# Autodesk Inventor assembly: Inner_Components
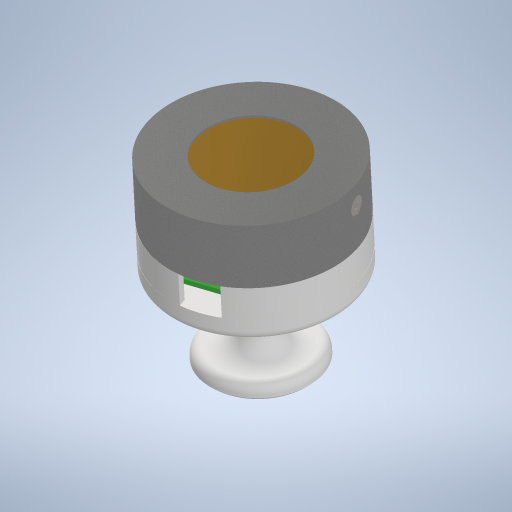
[picture p0: Inventor's stored thumbnail of the model, 512x512]
Saved by Autodesk Inventor 2023 (Build 270158000, 158)
## iProperties
Created: 2023-02-27
Part Number: Inner_Components
Document SubType Name: Assembly
Designer: maste
Author: maste
## Documents named in this file (9)
- C:\Users\maste\Documents\GitHub\Remote-Stethoscope\3D_models\ThonkLabs 1ne\SurfaceContact\Inner_Components.iam
- C:\Users\maste\Documents\GitHub\Remote-Stethoscope\3D_models\ThonkLabs 1ne\SurfaceContact\PiezoMount.ipt
- C:\Users\maste\Documents\GitHub\Remote-Stethoscope\3D_models\ThonkLabs 1ne\SurfaceContact\Piezo.ipt
- C:\Users\maste\Documents\GitHub\Remote-Stethoscope\3D_models\ThonkLabs 1ne\SurfaceContact\Diaphragm_lock.ipt
- C:\Users\maste\Documents\GitHub\Remote-Stethoscope\3D_models\ThonkLabs 1ne\SurfaceContact\holding_socket.ipt
- C:\Users\maste\Documents\GitHub\Remote-Stethoscope\3D_models\ThonkLabs 1ne\SurfaceContact\fasten_nut.ipt
- C:\Users\maste\Documents\GitHub\Remote-Stethoscope\3D_models\ThonkLabs 1ne\SurfaceContact\fasten_bolt.ipt
- C:\Users\maste\Documents\GitHub\Remote-Stethoscope\3D_models\xiao_rp2040\Seeed Studio XIAO RP2040 v26.iam
- C:\Users\maste\Documents\GitHub\Remote-Stethoscope\3D_models\ThonkLabs 1ne\SurfaceContact\Circuit_Board.ipt
## Components (14 placed, 8 different names)
1. PiezoMount:1 — Mate:33, Mate:36, Mate:37, Mate:39, Mate:41, Mate:44, Mate:48, Mate:49, Mate:50, Mate:51, Mate:53, Mate:54, Mate:56, Mate:57, Mate:58, Mate:59, Mate:60, Mate:61
2. Piezo:1 — Mate:46, Mate:47
3. Diaphragm_lock:1 — Mate:46, Mate:47, Mate:60, Mate:61
4. holding_socket:1 — Mate:58, Mate:59
5. fasten_nut:1 — Mate:52, Mate:53
6. fasten_nut:2 — Mate:55, Mate:56
7. fasten_bolt:1 — Mate:52, Mate:54
8. fasten_bolt:2 — Mate:55, Mate:57
9. fasten_nut:3 — Mate:41
10. fasten_nut:4 — Mate:48, Mate:49
11. fasten_bolt:3 — Mate:50, Mate:51
12. fasten_bolt:4 — Mate:39, Mate:44
13. Seeed Studio XIAO RP2040 v26:1 [sub-assembly] — Mate:34, Flush:1, Flush:2
14. Circuit_Board:1 — Mate:33, Mate:34, Flush:1, Flush:2, Mate:36, Mate:37
## Relationships (25: Mate 23, Flush 2)
- Mate:33 (3 mm): PiezoMount:1 ↔ Circuit_Board:1
- Mate:34 (3 mm): Seeed Studio XIAO RP2040 v26:1 ↔ Circuit_Board:1
- Flush:1: Seeed Studio XIAO RP2040 v26:1 ↔ Circuit_Board:1
- Flush:2 (7.8 mm): Seeed Studio XIAO RP2040 v26:1 ↔ Circuit_Board:1
- Mate:36: PiezoMount:1 ↔ Circuit_Board:1
- Mate:37: PiezoMount:1 ↔ Circuit_Board:1
- Mate:39: PiezoMount:1 ↔ fasten_bolt:4
- Mate:41: PiezoMount:1 ↔ fasten_nut:3
- Mate:44: PiezoMount:1 ↔ fasten_bolt:4
- Mate:46: Piezo:1 ↔ Diaphragm_lock:1
- Mate:47: Piezo:1 ↔ Diaphragm_lock:1
- Mate:48: PiezoMount:1 ↔ fasten_nut:4
- Mate:49: PiezoMount:1 ↔ fasten_nut:4
- Mate:50: PiezoMount:1 ↔ fasten_bolt:3
- Mate:51: PiezoMount:1 ↔ fasten_bolt:3
- Mate:52: fasten_nut:1 ↔ fasten_bolt:1
- Mate:53: PiezoMount:1 ↔ fasten_nut:1
- Mate:54: PiezoMount:1 ↔ fasten_bolt:1
- Mate:55: fasten_nut:2 ↔ fasten_bolt:2
- Mate:56: PiezoMount:1 ↔ fasten_nut:2
- Mate:57: PiezoMount:1 ↔ fasten_bolt:2
- Mate:58: PiezoMount:1 ↔ holding_socket:1
- Mate:59: PiezoMount:1 ↔ holding_socket:1
- Mate:60: PiezoMount:1 ↔ Diaphragm_lock:1
- Mate:61: PiezoMount:1 ↔ Diaphragm_lock:1
